# Autodesk Inventor assembly: InhalationAssembly
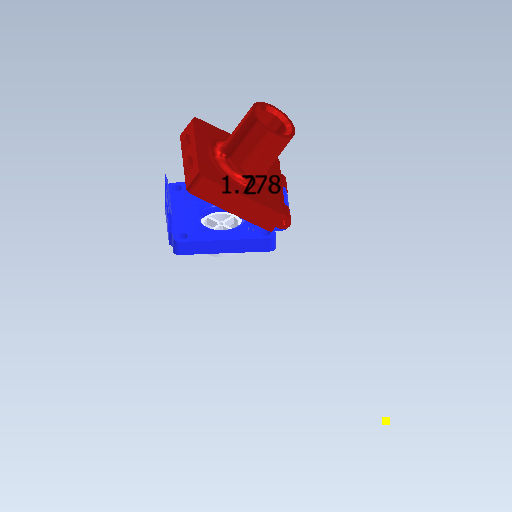
[picture p0: Inventor's stored thumbnail of the model, 512x512]
Saved by Autodesk Inventor 2020 (Build 240168000, 168)
## iProperties
Created: 2020-04-09
Part Number: InhalationAssembly
Document SubType Name: Assembly
Designer: Simon
Author: Simon
## Documents named in this file (4)
- \\Mac\Home\Desktop\3D\Breeze thing\Filter housing with o ring\InhalationAssembly.iam
- \\Mac\Home\Desktop\3D\Breeze thing\Filter housing with o ring\inhelationFilterHousing.iam
- \\Mac\Home\Desktop\3D\Breeze thing\Filter housing with o ring\clip.ipt
- \\Mac\Home\Desktop\3D\Breeze thing\Filter housing with o ring\filter_connector v1 (1).ipt
## Components (3 placed, 3 different names)
1. inhelationFilterHousing:1 [sub-assembly] — Mate:1, Mate:2, Mate:3, Mate:4, Mate:5
2. clip:1 — Mate:1, Mate:2, Mate:3
3. filter_connector v1 (1):1 — Mate:4, Mate:5
## Relationships (5: Mate 5)
- Mate:1: inhelationFilterHousing:1 ↔ clip:1
- Mate:2: inhelationFilterHousing:1 ↔ clip:1
- Mate:3: inhelationFilterHousing:1 ↔ clip:1
- Mate:4: inhelationFilterHousing:1 ↔ filter_connector v1 (1):1
- Mate:5 (0.25 mm): inhelationFilterHousing:1 ↔ filter_connector v1 (1):1
